# Autodesk Inventor assembly: Hinge
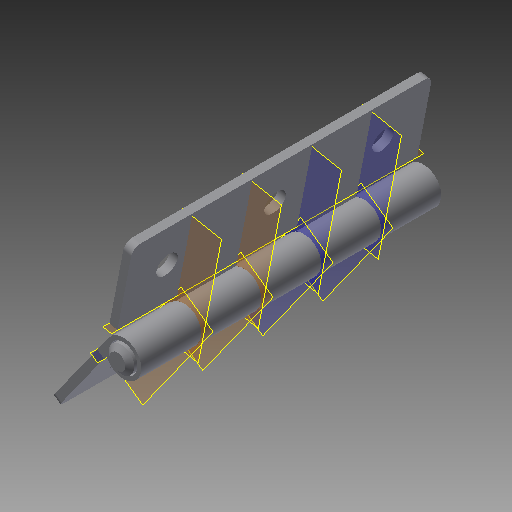
[picture p0: Inventor's stored thumbnail of the model, 512x512]
Saved by Autodesk Inventor 2019 (Build 230136000, 136)
## iProperties
Created: 2019-04-07
Part Number: Hinge
Material: 일반
Document SubType Name: Assembly
Designer: hinmo
Author: hinmo
## Documents named in this file (4)
- C:\Users\hinmo\Documents\Inventor\Projects\2019_CapstoneDesign\Hinge.iam
- C:\Users\hinmo\Documents\Inventor\Projects\2019_CapstoneDesign\Hinge_Part1.ipt
- C:\Users\hinmo\Documents\Inventor\Projects\2019_CapstoneDesign\Hinge_Part2.ipt
- C:\Users\hinmo\Documents\Inventor\Projects\2019_CapstoneDesign\Hinge_Poll.ipt
## Components (3 placed, 3 different names)
1. Hinge_Part1:1 — 메이트:1, 메이트:2
2. Hinge_Part2:1 — 메이트:1, 메이트:2, 메이트:3, 메이트:4
3. Hinge_Poll:1 — 메이트:3, 메이트:4
## Relationships (4: Mate 4)
- 메이트:1 [Mate]: Hinge_Part1:1 ↔ Hinge_Part2:1
- 메이트:2 [Mate]: Hinge_Part1:1 ↔ Hinge_Part2:1
- 메이트:3 [Mate]: Hinge_Part2:1 ↔ Hinge_Poll:1
- 메이트:4 [Mate] (0.5 mm): Hinge_Part2:1 ↔ Hinge_Poll:1
